# Autodesk Inventor assembly: 00_XY_stage-CHUO_SEIKI_LD-647-R1
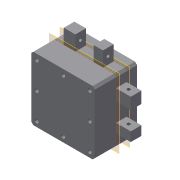
[picture p0: Inventor's stored thumbnail of the model, 180x180]
Saved by Autodesk Inventor 2019 (Build 230136000, 136)
## iProperties
Created: 2019-05-02
Part Number: 00_XY_stage-CHUO_SEIKI_LD-647-R1
Document SubType Name: Assembly
Designer: diederichbenedict
Author: diederichbenedict
## Documents named in this file (4)
- C:\Users\diederichbenedict\Dropbox\Dokumente\Promotion\PROJECTS\STORMoChip\INVENTOR\Nanoscopy-on-a-cheap\00_XY_stage-CHUO_SEIKI_LD-647-R1.iam
- C:\Users\diederichbenedict\Dropbox\Dokumente\Promotion\PROJECTS\STORMoChip\INVENTOR\Nanoscopy-on-a-cheap\00_XY_stage-CHUO_SEIKI_LD-647-R1-Top.ipt
- C:\Users\diederichbenedict\Dropbox\Dokumente\Promotion\PROJECTS\STORMoChip\INVENTOR\Nanoscopy-on-a-cheap\00_XY_stage-CHUO_SEIKI_LD-647-R1-Middle.ipt
- C:\Users\diederichbenedict\Dropbox\Dokumente\Promotion\PROJECTS\STORMoChip\INVENTOR\Nanoscopy-on-a-cheap\00_XY_stage-CHUO_SEIKI_LD-647-R1-Bottom.ipt
## Components (3 placed, 3 different names)
1. 00_XY_stage-CHUO_SEIKI_LD-647-R1-Top:1 — Flush:1, Flush:2, Mate:1
2. 00_XY_stage-CHUO_SEIKI_LD-647-R1-Middle:1 — Flush:1, Flush:2, Flush:3, Flush:4, Mate:1
3. 00_XY_stage-CHUO_SEIKI_LD-647-R1-Bottom:1 — Flush:3, Flush:4
## Relationships (5: Flush 4, Mate 1)
- Flush:1: 00_XY_stage-CHUO_SEIKI_LD-647-R1-Top:1 ↔ 00_XY_stage-CHUO_SEIKI_LD-647-R1-Middle:1
- Flush:2: 00_XY_stage-CHUO_SEIKI_LD-647-R1-Top:1 ↔ 00_XY_stage-CHUO_SEIKI_LD-647-R1-Middle:1
- Flush:3: 00_XY_stage-CHUO_SEIKI_LD-647-R1-Middle:1 ↔ 00_XY_stage-CHUO_SEIKI_LD-647-R1-Bottom:1
- Flush:4: 00_XY_stage-CHUO_SEIKI_LD-647-R1-Middle:1 ↔ 00_XY_stage-CHUO_SEIKI_LD-647-R1-Bottom:1
- Mate:1: 00_XY_stage-CHUO_SEIKI_LD-647-R1-Top:1 ↔ 00_XY_stage-CHUO_SEIKI_LD-647-R1-Middle:1
